# Autodesk Inventor assembly: Printer Frame Assembly RevII
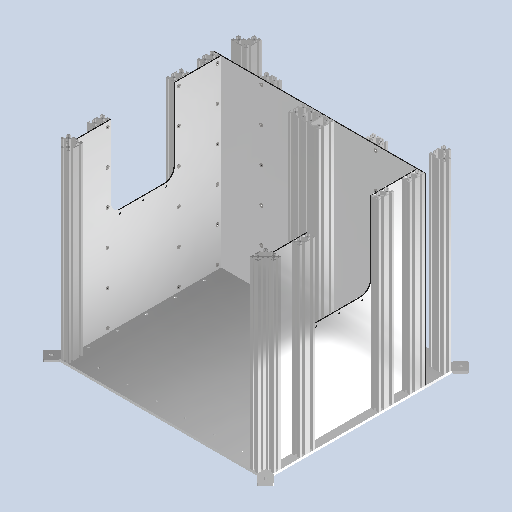
[picture p0: Inventor's stored thumbnail of the model, 512x512]
Saved by Autodesk Inventor 2024 (Build 280153000, 153)
## iProperties
Created: 2024-10-26
Part Number: Printer Frame Assembly RevII
Document SubType Name: Assembly
Designer: Ishaan
Author: Ishaan
## Documents named in this file (9)
- E:\Projects\Axiom--IDEX-3D-Printer\CAD\02 - Frame\Printer Frame Assembly RevII.iam
- E:\Projects\Axiom--IDEX-3D-Printer\CAD\02 - Frame\Printer Base Plate RevII.ipt
- E:\Projects\Axiom--IDEX-3D-Printer\CAD\00 - COTS Components\Hardware\Low Profile M5x12.ipt
- E:\Projects\Axiom--IDEX-3D-Printer\CAD\08 - Side Panelling\Internal Rear Panel Assembly.iam
- E:\Projects\Axiom--IDEX-3D-Printer\CAD\08 - Side Panelling\Left Internal Side Panel Assembly.iam
- E:\Projects\Axiom--IDEX-3D-Printer\CAD\08 - Side Panelling\Right Internal Side Panel Assembly.iam
- E:\Projects\Axiom--IDEX-3D-Printer\CAD\00 - COTS Components\4040 Vertical L Extrusions\HFS5-404020-475-SC.ipt
- E:\Projects\Axiom--IDEX-3D-Printer\CAD\00 - COTS Components\4080 Z-rail Extrusion\HFSP5-4080-475.ipt
- E:\Projects\Axiom--IDEX-3D-Printer\CAD\00 - COTS Components\2040 Vertical Extrusions\HFS5-2040-475-SC.ipt
## Components (49 placed, 8 different names)
1. Printer Base Plate RevII:1 — Mate:2, Mate:3, Mate:7
2. HFS5-404020-475-SC:1
3. HFS5-404020-475-SC:2
4. HFS5-404020-475-SC:3
5. HFS5-404020-475-SC:4
6. HFSP5-4080-475:1
7. HFS5-2040-475-SC:1
8. HFS5-2040-475-SC:2
9. HFS5-2040-475-SC:3
10. HFS5-2040-475-SC:4
11. HFS5-2040-475-SC:5
12. HFS5-2040-475-SC:6
13. HFS5-2040-475-SC:7
14. HFS5-2040-475-SC:8
15. Internal Rear Panel Assembly:1 [sub-assembly] — Mate:2
16. Left Internal Side Panel Assembly:1 [sub-assembly] — Mate:3
17. Right Internal Side Panel Assembly:1 [sub-assembly] — Mate:7
18. Low Profile M5x12:1
19. Low Profile M5x12:2
20. Low Profile M5x12:3
21. Low Profile M5x12:4
22. Low Profile M5x12:5
23. Low Profile M5x12:6
24. Low Profile M5x12:7
25. Low Profile M5x12:8
26. Low Profile M5x12:9
27. Low Profile M5x12:10
28. Low Profile M5x12:11
29. Low Profile M5x12:12
30. Low Profile M5x12:13
31. Low Profile M5x12:14
32. Low Profile M5x12:15
33. Low Profile M5x12:16
34. Low Profile M5x12:17
35. Low Profile M5x12:18
36. Low Profile M5x12:19
37. Low Profile M5x12:20
38. Low Profile M5x12:21
39. Low Profile M5x12:22
40. Low Profile M5x12:23
41. Low Profile M5x12:24
42. Low Profile M5x12:25
43. Low Profile M5x12:26
44. Low Profile M5x12:27
45. Low Profile M5x12:28
46. Low Profile M5x12:29
47. Low Profile M5x12:30
48. Low Profile M5x12:31
49. Low Profile M5x12:32
## Relationships (75: Insert 64, Mate 7, Flush 4)
- [Insert]: Printer Base Plate RevII:1 ↔ HFS5-404020-475-SC:1
- [Insert]: Printer Base Plate RevII:1 ↔ HFS5-404020-475-SC:1
- [Insert]: Printer Base Plate RevII:1 ↔ HFS5-404020-475-SC:2
- [Insert]: Printer Base Plate RevII:1 ↔ HFS5-404020-475-SC:2
- [Insert]: Printer Base Plate RevII:1 ↔ HFS5-404020-475-SC:3
- [Insert]: Printer Base Plate RevII:1 ↔ HFS5-404020-475-SC:3
- [Insert]: Printer Base Plate RevII:1 ↔ HFS5-404020-475-SC:4
- [Insert]: Printer Base Plate RevII:1 ↔ HFS5-404020-475-SC:4
- [Insert]: Printer Base Plate RevII:1 ↔ HFSP5-4080-475:1
- [Insert]: Printer Base Plate RevII:1 ↔ HFSP5-4080-475:1
- [Insert]: Printer Base Plate RevII:1 ↔ HFSP5-4080-475:1
- [Insert]: Printer Base Plate RevII:1 ↔ HFSP5-4080-475:1
- [Insert]: Printer Base Plate RevII:1 ↔ HFSP5-4080-475:1
- [Insert]: Printer Base Plate RevII:1 ↔ HFSP5-4080-475:1
- [Insert]: Printer Base Plate RevII:1 ↔ HFSP5-4080-475:1
- [Insert]: Printer Base Plate RevII:1 ↔ HFSP5-4080-475:1
- [Insert]: Printer Base Plate RevII:1 ↔ HFS5-2040-475-SC:6
- [Insert]: Printer Base Plate RevII:1 ↔ HFS5-2040-475-SC:6
- [Insert]: Printer Base Plate RevII:1 ↔ HFS5-2040-475-SC:5
- [Insert]: Printer Base Plate RevII:1 ↔ HFS5-2040-475-SC:5
- [Insert]: Printer Base Plate RevII:1 ↔ HFS5-2040-475-SC:4
- [Insert]: Printer Base Plate RevII:1 ↔ HFS5-2040-475-SC:4
- [Insert]: Printer Base Plate RevII:1 ↔ HFS5-2040-475-SC:1
- [Insert]: Printer Base Plate RevII:1 ↔ HFS5-2040-475-SC:1
- [Insert]: Printer Base Plate RevII:1 ↔ HFS5-2040-475-SC:3
- [Insert]: Printer Base Plate RevII:1 ↔ HFS5-2040-475-SC:3
- [Insert]: Printer Base Plate RevII:1 ↔ HFS5-2040-475-SC:2
- [Insert]: Printer Base Plate RevII:1 ↔ HFS5-2040-475-SC:2
- [Insert]: Printer Base Plate RevII:1 ↔ HFS5-2040-475-SC:8
- [Insert]: Printer Base Plate RevII:1 ↔ HFS5-2040-475-SC:8
- [Insert]: Printer Base Plate RevII:1 ↔ HFS5-2040-475-SC:7
- [Insert]: Printer Base Plate RevII:1 ↔ HFS5-2040-475-SC:7
- [Insert]: Printer Base Plate RevII:1 ↔ Low Profile M5x12:23
- [Insert]: Printer Base Plate RevII:1 ↔ Low Profile M5x12:24
- [Insert]: Printer Base Plate RevII:1 ↔ Low Profile M5x12:25
- [Insert]: Printer Base Plate RevII:1 ↔ Low Profile M5x12:26
- [Insert]: Printer Base Plate RevII:1 ↔ Low Profile M5x12:27
- [Insert]: Printer Base Plate RevII:1 ↔ Low Profile M5x12:28
- [Insert]: Printer Base Plate RevII:1 ↔ Low Profile M5x12:29
- [Insert]: Printer Base Plate RevII:1 ↔ Low Profile M5x12:30
- [Insert]: Printer Base Plate RevII:1 ↔ Low Profile M5x12:31
- [Insert]: Printer Base Plate RevII:1 ↔ Low Profile M5x12:32
- [Insert]: Printer Base Plate RevII:1 ↔ Low Profile M5x12:22
- [Insert]: Printer Base Plate RevII:1 ↔ Low Profile M5x12:21
- [Insert]: Printer Base Plate RevII:1 ↔ Low Profile M5x12:20
- [Insert]: Printer Base Plate RevII:1 ↔ Low Profile M5x12:19
- [Insert]: Printer Base Plate RevII:1 ↔ Low Profile M5x12:18
- [Insert]: Printer Base Plate RevII:1 ↔ Low Profile M5x12:17
- [Insert]: Printer Base Plate RevII:1 ↔ Low Profile M5x12:16
- [Insert]: Printer Base Plate RevII:1 ↔ Low Profile M5x12:15
- [Insert]: Printer Base Plate RevII:1 ↔ Low Profile M5x12:14
- [Insert]: Printer Base Plate RevII:1 ↔ Low Profile M5x12:13
- [Insert]: Printer Base Plate RevII:1 ↔ Low Profile M5x12:12
- [Insert]: Printer Base Plate RevII:1 ↔ Low Profile M5x12:11
- [Insert]: Printer Base Plate RevII:1 ↔ Low Profile M5x12:1
- [Insert]: Printer Base Plate RevII:1 ↔ Low Profile M5x12:2
- [Insert]: Printer Base Plate RevII:1 ↔ Low Profile M5x12:3
- [Insert]: Printer Base Plate RevII:1 ↔ Low Profile M5x12:4
- [Insert]: Printer Base Plate RevII:1 ↔ Low Profile M5x12:5
- [Insert]: Printer Base Plate RevII:1 ↔ Low Profile M5x12:6
- [Insert]: Printer Base Plate RevII:1 ↔ Low Profile M5x12:7
- [Insert]: Printer Base Plate RevII:1 ↔ Low Profile M5x12:8
- [Insert]: Printer Base Plate RevII:1 ↔ Low Profile M5x12:9
- [Insert]: Printer Base Plate RevII:1 ↔ Low Profile M5x12:10
- [Mate]: HFSP5-4080-475:1 ↔ Internal Rear Panel Assembly:1
- [Flush] (-1 mm): HFS5-2040-475-SC:4 ↔ Internal Rear Panel Assembly:1
- Mate:2 (1 mm): Printer Base Plate RevII:1 ↔ Internal Rear Panel Assembly:1
- [Flush] (1 mm): HFS5-2040-475-SC:3 ↔ Internal Rear Panel Assembly:1
- Mate:3 (1 mm): Printer Base Plate RevII:1 ↔ Left Internal Side Panel Assembly:1
- [Flush] (1 mm): HFS5-2040-475-SC:3 ↔ Left Internal Side Panel Assembly:1
- [Mate]: HFS5-2040-475-SC:3 ↔ Left Internal Side Panel Assembly:1
- [Mate] (1 mm): HFS5-404020-475-SC:1 ↔ Left Internal Side Panel Assembly:1
- [Mate]: HFS5-2040-475-SC:5 ↔ Right Internal Side Panel Assembly:1
- Mate:7 (1 mm): Printer Base Plate RevII:1 ↔ Right Internal Side Panel Assembly:1
- [Flush] (1 mm): HFS5-2040-475-SC:4 ↔ Right Internal Side Panel Assembly:1
